# Autodesk Inventor assembly: Kolov2
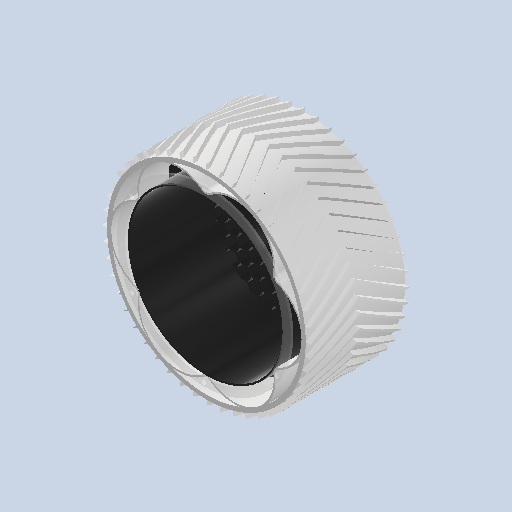
[picture p0: Inventor's stored thumbnail of the model, 512x512]
Saved by Autodesk Inventor 2025.3 (Build 293356000, 356)
## iProperties
Created: 2026-05-07
Part Number: Kolov2
Document SubType Name: Assembly
Designer: ksawe
Author: ksawe
## Documents named in this file (4)
- C:\Users\ksawe\OneDrive\Pulpit\Exomy v1\wersja3\Kolov2.iam
- C:\Users\ksawe\OneDrive\Pulpit\Exomy v1\wersja2\felga.ipt
- C:\Users\ksawe\OneDrive\Pulpit\Exomy v1\wersja3\opona_nowa.ipt
- C:\Users\ksawe\OneDrive\Pulpit\Exomy v1\wersja3\bead lock.ipt
## Components (4 placed, 3 different names)
1. felga:1 — Rigid:1, Rigid:2, Rigid:3
2. opona_nowa:1 — Rigid:1
3. bead lock:1 — Rigid:3
4. bead lock:2 — Rigid:2
## Relationships (3: WeldJoint 3)
- Rigid:1 [WeldJoint]: felga:1 ↔ opona_nowa:1
- Rigid:2 [WeldJoint] (-20 mm): felga:1 ↔ bead lock:2
- Rigid:3 [WeldJoint] (-20 mm): felga:1 ↔ bead lock:1
